# Autodesk Inventor assembly: Air puffs
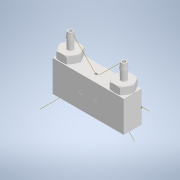
[picture p0: Inventor's stored thumbnail of the model, 180x180]
Saved by Autodesk Inventor 2021.2 (Build 252289000, 289)
## iProperties
Created: 2021-07-12
Part Number: Air puffs
Document SubType Name: Assembly
Designer: jl4459
Author: jl4459
## Documents named in this file (5)
- C:\Users\jl4459\Documents\Inventor\Training mini VR rig\Modules\Air puffs\Air puffs delivery.iam
- C:\Users\jl4459\Documents\Inventor\Training mini VR rig\Modules\Air puffs\Parts\air puffs delivery cover.ipt
- C:\Users\jl4459\Documents\Inventor\Training mini VR rig\Modules\Air puffs\Parts\air puffs delivery.ipt
- C:\Users\jl4459\Documents\Inventor\Training mini VR rig\Modules\Air puffs\Parts\91771A919_Passivated 18-8 Stainless Steel Phillips Flat Head Screw.ipt
- C:\Users\jl4459\Documents\Inventor\Training mini VR rig\Modules\Air puffs\Parts\5047K110_MOISTURE-RESISTANT ACETAL BARBED TUBE FITTING(1).ipt
## Components (6 placed, 4 different names)
1. air puffs delivery:1 — Mate:1, Mate:2, Insert:3, Insert:4
2. air puffs delivery cover:1 — Mate:1, Mate:2, Insert:1, Insert:2
3. 91771A919_Passivated 18-8 Stainless Steel Phillips Flat Head Screw:1 — Insert:1
4. 91771A919_Passivated 18-8 Stainless Steel Phillips Flat Head Screw:2 — Insert:2
5. 5047K110_MOISTURE-RESISTANT ACETAL BARBED TUBE FITTING(1):1 — Insert:3
6. 5047K110_MOISTURE-RESISTANT ACETAL BARBED TUBE FITTING(1):2 — Insert:4
## Relationships (6: Insert 4, Mate 2)
- Mate:1: air puffs delivery:1 ↔ air puffs delivery cover:1
- Mate:2: air puffs delivery:1 ↔ air puffs delivery cover:1
- Insert:1: air puffs delivery cover:1 ↔ 91771A919_Passivated 18-8 Stainless Steel Phillips Flat Head Screw:1
- Insert:2: air puffs delivery cover:1 ↔ 91771A919_Passivated 18-8 Stainless Steel Phillips Flat Head Screw:2
- Insert:3: air puffs delivery:1 ↔ 5047K110_MOISTURE-RESISTANT ACETAL BARBED TUBE FITTING(1):1
- Insert:4: air puffs delivery:1 ↔ 5047K110_MOISTURE-RESISTANT ACETAL BARBED TUBE FITTING(1):2
